# Autodesk Inventor assembly: Red Pump aa FINAL MODEL with drainage extension
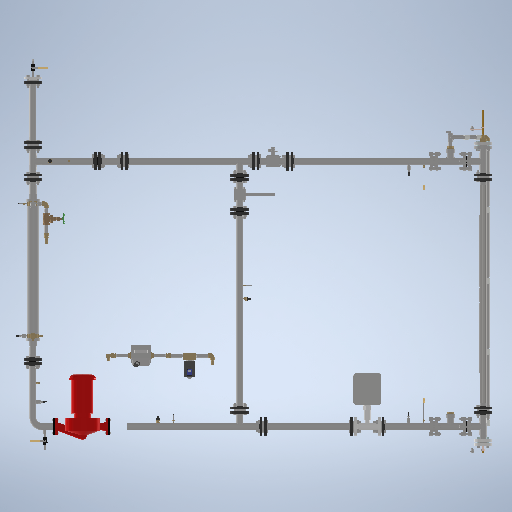
[picture p0: Inventor's stored thumbnail of the model, 512x512]
Saved by Autodesk Inventor 2027 (Build 310192000, 192)
## iProperties
Created: 2026-07-30
Part Number: Red Pump aa FINAL MODEL with drainage extension
Document SubType Name: Assembly
Designer: AdminForWorker
Title: aa FINAL MODEL with drainage extension v22
Author: AdminForWorker
## Documents named in this file (43)
- C:\Users\ig2\Desktop\SMR Thermal\thermal-loop\resources\v0.1.2\CAD\Inventor\aa FINAL MODEL with proportional valve\Red Pump aa FINAL MODEL with drainage extension.iam
- C:\Users\ig2\Desktop\SMR Thermal\thermal-loop\resources\v0.1.2\CAD\Inventor\aa FINAL MODEL with proportional valve\Average Flange Component (Larger Nut) v13.iam
- C:\Users\ig2\Desktop\SMR Thermal\thermal-loop\resources\v0.1.2\CAD\Inventor\aa FINAL MODEL with proportional valve\Average Flange Component (Larger Nut) v13_1.iam
- C:\Users\ig2\Desktop\SMR Thermal\thermal-loop\resources\v0.1.2\CAD\Inventor\aa FINAL MODEL with proportional valve\Flow-Tek Large Valve v6.ipt
- C:\Users\ig2\Desktop\SMR Thermal\thermal-loop\resources\v0.1.2\CAD\Inventor\aa FINAL MODEL with proportional valve\Average Flange Component (Larger Nut) v13_2.iam
- C:\Users\ig2\Desktop\SMR Thermal\thermal-loop\resources\v0.1.2\CAD\Inventor\aa FINAL MODEL with proportional valve\T pipe v3.ipt
- C:\Users\ig2\Desktop\SMR Thermal\thermal-loop\resources\v0.1.2\CAD\Inventor\aa FINAL MODEL with proportional valve\Average Flange Component (Larger Nut) v13_3.iam
- C:\Users\ig2\Desktop\SMR Thermal\thermal-loop\resources\v0.1.2\CAD\Inventor\aa FINAL MODEL with proportional valve\Average Flange Component (Larger Nut) v13_4.iam
- C:\Users\ig2\Desktop\SMR Thermal\thermal-loop\resources\v0.1.2\CAD\Inventor\aa FINAL MODEL with proportional valve\MC-II Flow Analyzer v7.iam
- C:\Users\ig2\Desktop\SMR Thermal\thermal-loop\resources\v0.1.2\CAD\Inventor\aa FINAL MODEL with proportional valve\Small I pipe v2.ipt
- C:\Users\ig2\Desktop\SMR Thermal\thermal-loop\resources\v0.1.2\CAD\Inventor\aa FINAL MODEL with proportional valve\Average Flange Component (Smaller Nut) v7.iam
- C:\Users\ig2\Desktop\SMR Thermal\thermal-loop\resources\v0.1.2\CAD\Inventor\aa FINAL MODEL with proportional valve\Pipe II v3.ipt
- C:\Users\ig2\Desktop\SMR Thermal\thermal-loop\resources\v0.1.2\CAD\Inventor\aa FINAL MODEL with proportional valve\Heater Connection Flange w_ rod v8.iam
- C:\Users\ig2\Desktop\SMR Thermal\thermal-loop\resources\v0.1.2\CAD\Inventor\aa FINAL MODEL with proportional valve\Pipe D v2.ipt
- C:\Users\ig2\Desktop\SMR Thermal\thermal-loop\resources\v0.1.2\CAD\Inventor\aa FINAL MODEL with proportional valve\Average Flange Component (Larger Nut) v13_5.iam
- C:\Users\ig2\Desktop\SMR Thermal\thermal-loop\resources\v0.1.2\CAD\Inventor\aa FINAL MODEL with proportional valve\Pipe C v2.ipt
- C:\Users\ig2\Desktop\SMR Thermal\thermal-loop\resources\v0.1.2\CAD\Inventor\aa FINAL MODEL with proportional valve\Average Flange Component (Larger Nut) v13_6.iam
- C:\Users\ig2\Desktop\SMR Thermal\thermal-loop\resources\v0.1.2\CAD\Inventor\aa FINAL MODEL with proportional valve\elbow 90_ pipe v5.ipt
- C:\Users\ig2\Desktop\SMR Thermal\thermal-loop\resources\v0.1.2\CAD\Inventor\aa FINAL MODEL with proportional valve\Average Flange Component (Larger Nut) v13_7.iam
- C:\Users\ig2\Desktop\SMR Thermal\thermal-loop\resources\v0.1.2\CAD\Inventor\aa FINAL MODEL with proportional valve\Short Piece for Tube v2.ipt
- C:\Users\ig2\Desktop\SMR Thermal\thermal-loop\resources\v0.1.2\CAD\Inventor\aa FINAL MODEL with proportional valve\Average Flange Component (Larger Nut) v13_8.iam
- C:\Users\ig2\Desktop\SMR Thermal\thermal-loop\resources\v0.1.2\CAD\Inventor\aa FINAL MODEL with proportional valve\Average Flange Component (Larger Nut) v13_9.iam
- C:\Users\ig2\Desktop\SMR Thermal\thermal-loop\resources\v0.1.2\CAD\Inventor\aa FINAL MODEL with proportional valve\Pipe A v4.ipt
- C:\Users\ig2\Desktop\SMR Thermal\thermal-loop\resources\v0.1.2\CAD\Inventor\aa FINAL MODEL with proportional valve\Air Exhaust Valve v11.iam
- C:\Users\ig2\Desktop\SMR Thermal\thermal-loop\resources\v0.1.2\CAD\Inventor\aa FINAL MODEL with proportional valve\Welded Extension Section Final v5.iam
- C:\Users\ig2\Desktop\SMR Thermal\thermal-loop\resources\v0.1.2\CAD\Inventor\aa FINAL MODEL with proportional valve\Average Flange Component (Smaller Nut) v7_1.iam
- C:\Users\ig2\Desktop\SMR Thermal\thermal-loop\resources\v0.1.2\CAD\Inventor\aa FINAL MODEL with proportional valve\Average Flange Component (Smaller Nut) v7_2.iam
- C:\Users\ig2\Desktop\SMR Thermal\thermal-loop\resources\v0.1.2\CAD\Inventor\aa FINAL MODEL with proportional valve\PipeAssembly1 v4.iam
- C:\Users\ig2\Desktop\SMR Thermal\thermal-loop\resources\v0.1.2\CAD\Inventor\aa FINAL MODEL with proportional valve\Welded Extension Section w_ relief v10.iam
- C:\Users\ig2\Desktop\SMR Thermal\thermal-loop\resources\v0.1.2\CAD\Inventor\aa FINAL MODEL with proportional valve\Top right non pressure relief v13.iam
- C:\Users\ig2\Desktop\SMR Thermal\thermal-loop\resources\v0.1.2\CAD\Inventor\aa FINAL MODEL with proportional valve\Extension plug v3.ipt
- C:\Users\ig2\Desktop\SMR Thermal\thermal-loop\resources\v0.1.2\CAD\Inventor\aa FINAL MODEL with proportional valve\Pipe J w_ sensors v3.iam
- C:\Users\ig2\Desktop\SMR Thermal\thermal-loop\resources\v0.1.2\CAD\Inventor\aa FINAL MODEL with proportional valve\Pipe E w_ sensors v2.iam
- C:\Users\ig2\Desktop\SMR Thermal\thermal-loop\resources\v0.1.2\CAD\Inventor\aa FINAL MODEL with proportional valve\Pipe B w_ sensors v1.iam
- C:\Users\ig2\Desktop\SMR Thermal\thermal-loop\resources\v0.1.2\CAD\Inventor\aa FINAL MODEL with proportional valve\Pipe F w_ sensors v1.iam
- C:\Users\ig2\Desktop\SMR Thermal\thermal-loop\resources\v0.1.2\CAD\Inventor\aa FINAL MODEL with proportional valve\Heat Exchanger w_ parts v8.iam
- C:\Users\ig2\Desktop\SMR Thermal\thermal-loop\resources\v0.1.2\CAD\Inventor\aa FINAL MODEL with proportional valve\Proportional valve setup v1.iam
- C:\Users\ig2\Desktop\SMR Thermal\thermal-loop\resources\v0.1.2\CAD\Inventor\aa FINAL MODEL with proportional valve\switch pipe valve v2.ipt
- C:\Users\ig2\Desktop\SMR Thermal\thermal-loop\resources\v0.1.2\CAD\Inventor\aa FINAL MODEL with proportional valve\Water Drainage for Red Pump.iam
- C:\Users\ig2\Desktop\SMR Thermal\thermal-loop\resources\v0.1.2\CAD\Inventor\aa FINAL MODEL with proportional valve\Red pump regular pipe to pump pipe connector v3.ipt
- C:\Users\ig2\Desktop\SMR Thermal\thermal-loop\resources\v0.1.2\CAD\Inventor\aa FINAL MODEL with proportional valve\Red Pump Pipe I w_ sensors v1.iam
- C:\Users\ig2\Desktop\SMR Thermal\thermal-loop\resources\v0.1.2\CAD\Inventor\aa FINAL MODEL with proportional valve\Red Pump Pipe H w_ sensors v1.iam
- C:\Users\ig2\Desktop\SMR Thermal\thermal-loop\resources\v0.1.2\CAD\Inventor\aa FINAL MODEL with proportional valve\Red Pump Assembly.iam
## Components (48 placed, 31 different names)
1. Average Flange Component (Larger Nut) v13:1 [sub-assembly]
2. Average Flange Component (Larger Nut) v13:2 [sub-assembly]
3. Flow-Tek Large Valve v6:1
4. Average Flange Component (Larger Nut) v13:3 [sub-assembly]
5. T pipe v3:2
6. Average Flange Component (Larger Nut) v13:4 [sub-assembly]
7. Average Flange Component (Larger Nut) v13:5 [sub-assembly]
8. Flow-Tek Large Valve v6:2
9. T pipe v3:3
10. T pipe v3:4
11. T pipe v3:5 — Rotational:2
12. MC-II Flow Analyzer v7:1 [sub-assembly]
13. Small I pipe v2:1
14. Average Flange Component (Smaller Nut) v7:3 [sub-assembly]
15. Pipe II v3:1
16. Heater Connection Flange w/ rod v8:1 [sub-assembly]
17. Pipe D v2:1
18. Average Flange Component (Larger Nut) v13:6 [sub-assembly]
19. Pipe C v2:1
20. Average Flange Component (Larger Nut) v13:7 [sub-assembly]
21. elbow 90* pipe v5:1 — Rigid:1, Rotational:8
22. Average Flange Component (Larger Nut) v13:8 [sub-assembly] — Rotational:7
23. Short Piece for Tube v2:1
24. Short Piece for Tube v2:2
25. Average Flange Component (Larger Nut) v13:9 [sub-assembly]
26. T pipe v3:6
27. Average Flange Component (Larger Nut) v13:10 [sub-assembly]
28. Pipe A v4:1
29. Air Exhaust Valve v11:1 [sub-assembly]
30. Welded Extension Section Final v5:2 [sub-assembly]
31. Average Flange Component (Smaller Nut) v7:4 [sub-assembly]
32. Average Flange Component (Smaller Nut) v7:5 [sub-assembly]
33. PipeAssembly1 v4:1 [sub-assembly]
34. Welded Extension Section w/ relief v10:1 [sub-assembly]
35. Top right non pressure relief v13:1 [sub-assembly]
36. Extension plug v3:1
37. Pipe J w/ sensors v3:1 [sub-assembly]
38. Pipe E w/ sensors v2:1 [sub-assembly]
39. Pipe B w/ sensors v1:1 [sub-assembly]
40. Pipe F w/ sensors v1:1 [sub-assembly]
41. Heat Exchanger w/ parts v8:1 [sub-assembly] — Rotational:1
42. Proportional valve setup v1:1 [sub-assembly]
43. switch pipe valve v2:1 — Rotational:1
44. Water Drainage for Red Pump:1 [sub-assembly] — Rigid:1, Rotational:9
45. Red pump regular pipe to pump pipe connector v3:1 — Rigid:2
46. Red Pump Pipe I w_ sensors v1:1 [sub-assembly] — Rotational:2, Rigid:2
47. Red Pump Pipe H w_ sensors v1:1 [sub-assembly] — Rotational:7, Rotational:8
48. Red Pump Assembly:1 [sub-assembly] — Rotational:9
## Relationships (7: RevoluteJoint 5, WeldJoint 2)
- Rotational:1 [RevoluteJoint]: Heat Exchanger w/ parts v8:1 ↔ switch pipe valve v2:1
- Rigid:1 [WeldJoint]: elbow 90* pipe v5:1 ↔ Water Drainage for Red Pump:1
- Rotational:2 [RevoluteJoint]: T pipe v3:5 ↔ Red Pump Pipe I w_ sensors v1:1
- Rotational:7 [RevoluteJoint]: Average Flange Component (Larger Nut) v13:8 ↔ Red Pump Pipe H w_ sensors v1:1
- Rotational:8 [RevoluteJoint]: elbow 90* pipe v5:1 ↔ Red Pump Pipe H w_ sensors v1:1
- Rigid:2 [WeldJoint]: Red pump regular pipe to pump pipe connector v3:1 ↔ Red Pump Pipe I w_ sensors v1:1
- Rotational:9 [RevoluteJoint]: Water Drainage for Red Pump:1 ↔ Red Pump Assembly:1
